# Autodesk Inventor assembly: Fr.wing_assy
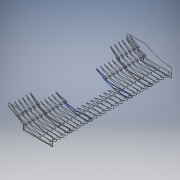
[picture p0: Inventor's stored thumbnail of the model, 180x180]
Saved by Autodesk Inventor 2018.2 (Build 222227000, 227)
## iProperties
Created: 2018-03-05
Part Number: Fr.wing_assy
Material: 一般
Document SubType Name: Assembly
Designer: ku_sk
Author: ku_sk
## Documents named in this file (8)
- C:\Users\ku_sk\Documents\Inventor\AeroCAD2018\設計\Fr.wing\製作用\Fr.wing_assy.iam
- C:\Users\ku_sk\Documents\Inventor\AeroCAD2018\設計\Fr.wing\製作用\parts\mainflap_side\mainflap_side.iam
- C:\Users\ku_sk\Documents\Inventor\AeroCAD2018\設計\Fr.wing\製作用\parts\mainflap_center\mainflap_center.iam
- C:\Users\ku_sk\Documents\Inventor\AeroCAD2018\設計\Fr.wing\製作用\parts\subflap\subflap.iam
- C:\Users\ku_sk\Documents\Inventor\AeroCAD2018\設計\Fr.wing\製作用\parts\bracket1.ipt
- C:\Users\ku_sk\Documents\Inventor\AeroCAD2018\設計\Fr.wing\製作用\parts\bracket2.ipt
- C:\Users\ku_sk\Documents\Inventor\AeroCAD2018\設計\Fr.wing\製作用\parts\endplate.ipt
- C:\Users\ku_sk\Documents\Inventor\AeroCAD2018\設計\Fr.wing\製作用\parts\endplate1.ipt
## Components (17 placed, 7 different names)
1. mainflap_center:1 [sub-assembly] — フラッシュ:1, メイト:1, メイト:2, メイト:3, メイト:4, メイト:5, メイト:6, メイト:7, 角度:1
2. mainflap_side:1 [sub-assembly] — メイト:2, メイト:4, メイト:7, メイト:8, メイト:9, メイト:10, フラッシュ:2, メイト:27, メイト:28, メイト:29, メイト:40, メイト:41
3. mainflap_side:2 [sub-assembly] — メイト:3, メイト:5, メイト:6, メイト:11, メイト:12, メイト:13, フラッシュ:4, メイト:24, メイト:25, メイト:26, メイト:34
4. mainflap_side:3 [sub-assembly] — メイト:8, メイト:9, メイト:10, フラッシュ:3, メイト:39, メイト:45
5. mainflap_side:4 [sub-assembly] — メイト:11, メイト:12, メイト:13, フラッシュ:5, メイト:35, メイト:36, メイト:44
6. subflap:1 [sub-assembly] — メイト:14, メイト:15, メイト:19, フラッシュ:2, メイト:20, メイト:21, メイト:30, メイト:31
7. subflap:2 [sub-assembly] — メイト:14, メイト:15, メイト:19, フラッシュ:3, フラッシュ:7
8. subflap:3 [sub-assembly] — メイト:22, メイト:23, フラッシュ:7, メイト:42, メイト:43
9. subflap:4 [sub-assembly] — メイト:16, メイト:17, メイト:18, フラッシュ:4, メイト:20, メイト:21, メイト:32, メイト:33
10. subflap:5 [sub-assembly] — メイト:16, メイト:17, メイト:18, フラッシュ:5, フラッシュ:6
11. subflap:6 [sub-assembly] — メイト:22, メイト:23, フラッシュ:6, メイト:37, メイト:38
12. bracket1:1 — メイト:24, メイト:25, メイト:26, メイト:32, メイト:33
13. bracket1:2 — メイト:27, メイト:28, メイト:29, メイト:30, メイト:31
14. bracket2:1 — メイト:34, メイト:35, メイト:36, メイト:37, メイト:38
15. bracket2:2 — メイト:39, メイト:40, メイト:41, メイト:42, メイト:43
16. endplate:1 — メイト:44, フラッシュ:8, フラッシュ:9
17. endplate1:1 — メイト:45, フラッシュ:8, フラッシュ:9
## Relationships (55: Mate 45, Flush 9, Angle 1)
- フラッシュ:1 [Flush]: mainflap_center:1
- メイト:1 [Mate]: mainflap_center:1
- メイト:2 [Mate] (4 mm): mainflap_center:1 ↔ mainflap_side:1
- メイト:3 [Mate] (4 mm): mainflap_center:1 ↔ mainflap_side:2
- メイト:4 [Mate]: mainflap_center:1 ↔ mainflap_side:1
- メイト:5 [Mate]: mainflap_center:1 ↔ mainflap_side:2
- メイト:6 [Mate]: mainflap_center:1 ↔ mainflap_side:2
- メイト:7 [Mate]: mainflap_center:1 ↔ mainflap_side:1
- メイト:8 [Mate] (4 mm): mainflap_side:1 ↔ mainflap_side:3
- メイト:9 [Mate]: mainflap_side:1 ↔ mainflap_side:3
- メイト:10 [Mate]: mainflap_side:1 ↔ mainflap_side:3
- メイト:11 [Mate] (4 mm): mainflap_side:2 ↔ mainflap_side:4
- メイト:12 [Mate]: mainflap_side:2 ↔ mainflap_side:4
- メイト:13 [Mate]: mainflap_side:2 ↔ mainflap_side:4
- メイト:14 [Mate]: subflap:1 ↔ subflap:2
- メイト:15 [Mate]: subflap:1 ↔ subflap:2
- メイト:16 [Mate] (4 mm): subflap:4 ↔ subflap:5
- メイト:17 [Mate]: subflap:4 ↔ subflap:5
- メイト:18 [Mate]: subflap:4 ↔ subflap:5
- メイト:19 [Mate] (4 mm): subflap:1 ↔ subflap:2
- フラッシュ:2 [Flush]: mainflap_side:1 ↔ subflap:1
- フラッシュ:3 [Flush]: mainflap_side:3 ↔ subflap:2
- フラッシュ:4 [Flush]: mainflap_side:2 ↔ subflap:4
- フラッシュ:5 [Flush]: mainflap_side:4 ↔ subflap:5
- メイト:20 [Mate]: subflap:1 ↔ subflap:4
- メイト:21 [Mate]: subflap:1 ↔ subflap:4
- メイト:22 [Mate]: subflap:3 ↔ subflap:6
- メイト:23 [Mate]: subflap:3 ↔ subflap:6
- フラッシュ:6 [Flush]: subflap:5 ↔ subflap:6
- フラッシュ:7 [Flush]: subflap:2 ↔ subflap:3
- メイト:24 [Mate]: mainflap_side:2 ↔ bracket1:1
- メイト:25 [Mate]: mainflap_side:2 ↔ bracket1:1
- メイト:26 [Mate]: mainflap_side:2 ↔ bracket1:1
- メイト:27 [Mate]: mainflap_side:1 ↔ bracket1:2
- メイト:28 [Mate]: mainflap_side:1 ↔ bracket1:2
- メイト:29 [Mate]: mainflap_side:1 ↔ bracket1:2
- メイト:30 [Mate]: subflap:1 ↔ bracket1:2
- メイト:31 [Mate]: subflap:1 ↔ bracket1:2
- メイト:32 [Mate]: subflap:4 ↔ bracket1:1
- メイト:33 [Mate]: subflap:4 ↔ bracket1:1
- メイト:34 [Mate]: mainflap_side:2 ↔ bracket2:1
- メイト:35 [Mate]: mainflap_side:4 ↔ bracket2:1
- メイト:36 [Mate]: mainflap_side:4 ↔ bracket2:1
- メイト:37 [Mate]: subflap:6 ↔ bracket2:1
- メイト:38 [Mate]: subflap:6 ↔ bracket2:1
- メイト:39 [Mate]: mainflap_side:3 ↔ bracket2:2
- メイト:40 [Mate]: mainflap_side:1 ↔ bracket2:2
- メイト:41 [Mate]: mainflap_side:1 ↔ bracket2:2
- メイト:42 [Mate]: subflap:3 ↔ bracket2:2
- メイト:43 [Mate]: subflap:3 ↔ bracket2:2
- メイト:44 [Mate]: mainflap_side:4 ↔ endplate:1
- メイト:45 [Mate]: mainflap_side:3 ↔ endplate1:1
- フラッシュ:8 [Flush]: endplate:1 ↔ endplate1:1
- フラッシュ:9 [Flush]: endplate:1 ↔ endplate1:1
- 角度:1 [Angle] (2 deg): mainflap_center:1
